# Autodesk Inventor assembly: Door with Laguna Fast50
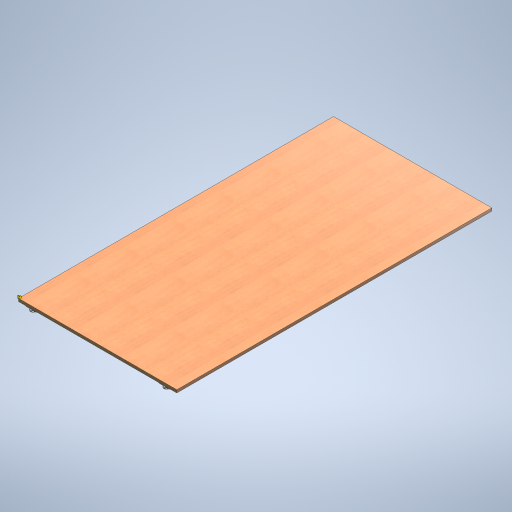
[picture p0: Inventor's stored thumbnail of the model, 512x512]
Saved by Autodesk Inventor 2024 (Build 280153000, 153)
## iProperties
RuleStatus: InUse
Created: 2014-10-21
Part Number: Door with Laguna Fast50
Document SubType Name: Assembly
Designer: G. Kazokaitis
Author: G. Kazokaitis
## Documents named in this file (6)
- C:\W4INV 2024 Design\iBOX LIBRARY\Door systems\Laguna Fast50 System\Door with Laguna Fast50.iam
- C:\W4INV 2024 Design\iBOX LIBRARY\Door systems\Laguna Fast50 System\Parts\Door.ipt
- C:\W4INV 2024 Design\iBOX LIBRARY\Door systems\Laguna Fast50 System\Parts\Door skeleton.ipt
- C:\W4INV 2024 Design\iBOX LIBRARY\Door systems\Laguna Fast50 System\Parts\Wheel with plate.ipt
- C:\W4INV 2024 Design\iBOX LIBRARY\Door systems\Laguna Fast50 System\Parts\Top plate.ipt
- C:\W4INV 2024 Design\iBOX LIBRARY\Door systems\Laguna Fast50 System\Parts\Fixing plate.ipt
## Components (8 placed, 8 different names)
1. @Skeleton — Flush:15
2. Door:1 — Door Planar Plane:6, Flush:15, Mate:14, Mate:15, Mate:16, Flush:17, Mate:17, Flush:18, Mate:18, Flush:19, Mate:19, Flush:20, Mate:20, Mate:21
3. @Wheel with plate Left side — Mate:14, Mate:17, Flush:18
4. @Wheel with plate Right side — Mate:15, Mate:16, Flush:17
5. @Top plate Right side — Mate:18, Flush:19, Mate:19, Flush:24, Flush:25, Flush:26
6. @Top plate Left side — Flush:20, Mate:20, Mate:21, Flush:21, Flush:22, Flush:23
7. @Fixing plate Left — Flush:21, Flush:22, Flush:23
8. @Fixing plate Right — Door Planar Plane:6, Flush:24, Flush:25, Flush:26
## Relationships (20: Flush 12, Mate 8)
- Door Planar Plane:6 [Flush] (-19 mm): Door:1 ↔ @Fixing plate Right
- Flush:15: @Skeleton ↔ Door:1
- Mate:14 (-79 mm): Door:1 ↔ @Wheel with plate Left side
- Mate:15 (-79 mm): Door:1 ↔ @Wheel with plate Right side
- Mate:16: Door:1 ↔ @Wheel with plate Right side
- Flush:17: Door:1 ↔ @Wheel with plate Right side
- Mate:17: Door:1 ↔ @Wheel with plate Left side
- Flush:18: Door:1 ↔ @Wheel with plate Left side
- Mate:18 (-66 mm): Door:1 ↔ @Top plate Right side
- Flush:19 (-7 mm): Door:1 ↔ @Top plate Right side
- Mate:19: Door:1 ↔ @Top plate Right side
- Flush:20 (-7 mm): Door:1 ↔ @Top plate Left side
- Mate:20: Door:1 ↔ @Top plate Left side
- Mate:21 (-66 mm): Door:1 ↔ @Top plate Left side
- Flush:21 (2 mm): @Top plate Left side ↔ @Fixing plate Left
- Flush:22: @Top plate Left side ↔ @Fixing plate Left
- Flush:23 (-4.75 mm): @Top plate Left side ↔ @Fixing plate Left
- Flush:24 (-2 mm): @Top plate Right side ↔ @Fixing plate Right
- Flush:25 (4.75 mm): @Top plate Right side ↔ @Fixing plate Right
- Flush:26: @Top plate Right side ↔ @Fixing plate Right
